# Autodesk Inventor assembly: Assembly_base
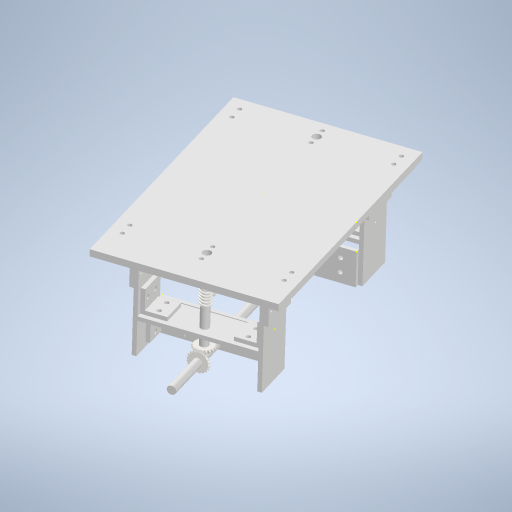
[picture p0: Inventor's stored thumbnail of the model, 512x512]
Saved by Autodesk Inventor 2023 (Build 270158000, 158)
## iProperties
Created: 2023-02-09
Part Number: Assembly_base
Document SubType Name: Assembly
Designer: deepa
Author: deepa
## Documents named in this file (14)
- C:\Users\Nikhil\Documents\GitHub\Ta_Project_Group27\Assembly_base.iam
- C:\Users\Nikhil\Documents\GitHub\Ta_Project_Group27\Base Plate.ipt
- C:\Users\Nikhil\Documents\GitHub\Ta_Project_Group27\Base_Connector1.ipt
- C:\Users\Nikhil\Documents\GitHub\Ta_Project_Group27\Base_Connector2.ipt
- C:\Users\Nikhil\Documents\GitHub\Ta_Project_Group27\Side_Plate1.ipt
- C:\Users\Nikhil\Documents\GitHub\Ta_Project_Group27\Side_plate2.ipt
- C:\Users\Nikhil\Documents\GitHub\Ta_Project_Group27\support plate 2.ipt
- C:\Users\Nikhil\Documents\GitHub\Ta_Project_Group27\Normal_Connector.ipt
- C:\Users\Nikhil\Documents\GitHub\Ta_Project_Group27\support plate 3.ipt
- C:\Users\Nikhil\Documents\GitHub\Ta_Project_Group27\rod_450mm.ipt
- C:\Users\Nikhil\Documents\GitHub\Ta_Project_Group27\shaft_120mm.ipt
- C:\Users\Nikhil\Documents\GitHub\Ta_Project_Group27\Assembly_base\Design Accelerator\Bevel Gears1.iam
- C:\Users\Nikhil\Documents\GitHub\Ta_Project_Group27\Assembly_base\Design Accelerator\Bevel Gears2.iam
- C:\Users\Nikhil\Documents\GitHub\Ta_Project_Group27\Assembly_base\Design Accelerator\Worm Gears4.iam
## Components (28 placed, 12 different names)
1. Base Plate:1 — Mate:1, Mate:2, Mate:3, Mate:4, Mate:5, Mate:6, Mate:7, Mate:8, Mate:9, Mate:10, Mate:11, Mate:12, Mate:13, Mate:14, Mate:15, Mate:16, Mate:21, Mate:74, Mate:75
2. Base_Connector1:1 — Mate:1, Mate:2, Mate:3, Mate:22, Mate:23
3. Base_Connector1:2 — Mate:4, Mate:5, Mate:6, Mate:26, Mate:32
4. Base_Connector2:1 — Mate:7, Mate:11, Mate:12, Mate:18, Mate:19
5. Base_Connector2:2 — Mate:8, Mate:9, Mate:10, Mate:24, Mate:25
6. Side_Plate1:1 — Mate:14, Mate:21, Mate:22, Mate:23, Mate:40, Flush:1, Mate:54
7. Side_plate2:1 — Mate:13, Mate:18, Mate:19, Flush:2, Mate:45, Mate:46, Mate:72
8. Side_Plate1:2 — Mate:15, Mate:24, Mate:25, Mate:39, Flush:3, Mate:51
9. Side_plate2:2 — Mate:16, Mate:26, Mate:32, Flush:4, Mate:57
10. support plate 2:1 — Mate:36, Mate:37, Mate:38, Mate:40, Flush:1, Mate:53, Mate:73
11. Normal_Connector:1 — Mate:36, Mate:38, Mate:39, Flush:5
12. Normal_Connector:2 — Mate:37, Mate:54, Flush:6
13. support plate 2:2 — Flush:2, Mate:46, Mate:56, Mate:58
14. Normal_Connector:3 — Mate:45, Flush:6
15. Normal_Connector:4 — Mate:57, Mate:58, Flush:5
16. support plate 3:1 — Flush:4, Mate:56, Mate:61, Mate:62, Mate:69, Mate:70, Mate:71
17. support plate 3:2 — Flush:3, Mate:51, Mate:53, Mate:60, Mate:63, Mate:64, Mate:65, Mate:66, Mate:67, Mate:68
18. Normal_Connector:5 — Mate:66, Mate:67, Mate:68
19. Normal_Connector:6 — Mate:60, Mate:61, Mate:62
20. Normal_Connector:7 — Mate:63, Mate:64, Mate:65
21. Normal_Connector:8 — Mate:69, Mate:70, Mate:71, Mate:72
22. rod_450mm:1 — Mate:73, Mate:76, Mate:77
23. shaft_120mm:1 — Mate:75, Mate:78, Mate:81
24. shaft_120mm:2 — Mate:74, Mate:79, Mate:80
25. Bevel Gears:1 [sub-assembly] — Mate:76, Mate:79
26. Bevel Gears:2 [sub-assembly] — Mate:77, Mate:78
27. Worm Gears:5 [sub-assembly] — Mate:80, Mate:82
28. Worm Gears:6 [sub-assembly] — Mate:81, Mate:82
## Relationships (69: Mate 63, Flush 6)
- Mate:1: Base Plate:1 ↔ Base_Connector1:1
- Mate:2: Base Plate:1 ↔ Base_Connector1:1
- Mate:3: Base Plate:1 ↔ Base_Connector1:1
- Mate:4: Base Plate:1 ↔ Base_Connector1:2
- Mate:5: Base Plate:1 ↔ Base_Connector1:2
- Mate:6: Base Plate:1 ↔ Base_Connector1:2
- Mate:7: Base Plate:1 ↔ Base_Connector2:1
- Mate:8: Base Plate:1 ↔ Base_Connector2:2
- Mate:9: Base Plate:1 ↔ Base_Connector2:2
- Mate:10: Base Plate:1 ↔ Base_Connector2:2
- Mate:11: Base Plate:1 ↔ Base_Connector2:1
- Mate:12: Base Plate:1 ↔ Base_Connector2:1
- Mate:13: Base Plate:1 ↔ Side_plate2:1
- Mate:14: Base Plate:1 ↔ Side_Plate1:1
- Mate:15: Base Plate:1 ↔ Side_Plate1:2
- Mate:16: Base Plate:1 ↔ Side_plate2:2
- Mate:18: Base_Connector2:1 ↔ Side_plate2:1
- Mate:19: Base_Connector2:1 ↔ Side_plate2:1
- Mate:21: Base Plate:1 ↔ Side_Plate1:1
- Mate:22: Base_Connector1:1 ↔ Side_Plate1:1
- Mate:23: Base_Connector1:1 ↔ Side_Plate1:1
- Mate:24: Base_Connector2:2 ↔ Side_Plate1:2
- Mate:25: Base_Connector2:2 ↔ Side_Plate1:2
- Mate:26: Base_Connector1:2 ↔ Side_plate2:2
- Mate:32: Base_Connector1:2 ↔ Side_plate2:2
- Mate:36: support plate 2:1 ↔ Normal_Connector:1
- Mate:37: support plate 2:1 ↔ Normal_Connector:2
- Mate:38: support plate 2:1 ↔ Normal_Connector:1
- Mate:39: Side_Plate1:2 ↔ Normal_Connector:1
- Mate:40: Side_Plate1:1 ↔ support plate 2:1
- Flush:1: Side_Plate1:1 ↔ support plate 2:1
- [Mate]: support plate 2:2 ↔ Normal_Connector:3
- [Mate]: support plate 2:2 ↔ Normal_Connector:3
- Flush:2: Side_plate2:1 ↔ support plate 2:2
- Mate:45: Side_plate2:1 ↔ Normal_Connector:3
- Mate:46: Side_plate2:1 ↔ support plate 2:2
- Flush:3: Side_Plate1:2 ↔ support plate 3:2
- Mate:51: Side_Plate1:2 ↔ support plate 3:2
- Mate:53: support plate 2:1 ↔ support plate 3:2
- Mate:54: Side_Plate1:1 ↔ Normal_Connector:2
- Flush:4: Side_plate2:2 ↔ support plate 3:1
- Mate:56: support plate 2:2 ↔ support plate 3:1
- Mate:57: Side_plate2:2 ↔ Normal_Connector:4
- Mate:58: support plate 2:2 ↔ Normal_Connector:4
- Flush:5: Normal_Connector:1 ↔ Normal_Connector:4
- Flush:6: Normal_Connector:2 ↔ Normal_Connector:3
- Mate:60: support plate 3:2 ↔ Normal_Connector:6
- Mate:61: support plate 3:1 ↔ Normal_Connector:6
- Mate:62: support plate 3:1 ↔ Normal_Connector:6
- Mate:63: support plate 3:2 ↔ Normal_Connector:7
- Mate:64: support plate 3:2 ↔ Normal_Connector:7
- Mate:65: support plate 3:2 ↔ Normal_Connector:7
- Mate:66: support plate 3:2 ↔ Normal_Connector:5
- Mate:67: support plate 3:2 ↔ Normal_Connector:5
- Mate:68: support plate 3:2 ↔ Normal_Connector:5
- Mate:69: support plate 3:1 ↔ Normal_Connector:8
- Mate:70: support plate 3:1 ↔ Normal_Connector:8
- Mate:71: support plate 3:1 ↔ Normal_Connector:8
- Mate:72: Side_plate2:1 ↔ Normal_Connector:8
- Mate:73: support plate 2:1 ↔ rod_450mm:1
- Mate:74: Base Plate:1 ↔ shaft_120mm:2
- Mate:75: Base Plate:1 ↔ shaft_120mm:1
- Mate:76: rod_450mm:1 ↔ Bevel Gears:1
- Mate:77: rod_450mm:1 ↔ Bevel Gears:2
- Mate:78: shaft_120mm:1 ↔ Bevel Gears:2
- Mate:79: shaft_120mm:2 ↔ Bevel Gears:1
- Mate:80: shaft_120mm:2 ↔ Worm Gears:5
- Mate:81: shaft_120mm:1 ↔ Worm Gears:6
- Mate:82: Worm Gears:5 ↔ Worm Gears:6
## Named parameters: d58_d50 = 0 mm, d60_d53 = 0 mm
